# Autodesk Inventor assembly: am14u3LongWithCubeAndWinch
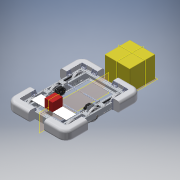
[picture p0: Inventor's stored thumbnail of the model, 180x180]
Saved by Autodesk Inventor 2018.2 (Build 222227000, 227)
## iProperties
Created: 2018-01-10
Part Number: am14u3LongWithCubeAndWinch
Document SubType Name: Assembly
Designer: steele
Author: steele
## Documents named in this file (5)
- D:\snobotics\CAD-Development\robSteele\2018-FRC\am14u3LongWithCubeAndWinch.iam
- D:\snobotics\CAD-Development\robSteele\2018-FRC\AM14U3 Long with Bumper\DB_DriveBaseLong_AM14U3_Bumpers and Battery Tray.iam
- D:\snobotics\CAD-Development\robSteele\2018-FRC\Field Elements\Cube-GE-18124.ipt
- D:\snobotics\CAD-Development\robSteele\2018-FRC\AluminumPlateForWinch.ipt
- D:\snobotics\CAD-Development\robSteele\2018-FRC\WinchVolume.ipt
## Components (4 placed, 4 different names)
1. DB_DriveBaseLong_AM14U3_Bumpers and Battery Tray:1 [sub-assembly] — Mate:1, Mate:2, Mate:3, Mate:4, Flush:2, Mate:5
2. Cube-GE-18124:1 — Mate:1, Flush:1, Mate:2
3. AluminumPlateForWinch:1 — Mate:3, Mate:4, Flush:2, Mate:6, Flush:3
4. WinchVolume:1 — Mate:5, Mate:6, Flush:3
## Relationships (9: Mate 6, Flush 3)
- Mate:1: DB_DriveBaseLong_AM14U3_Bumpers and Battery Tray:1 ↔ Cube-GE-18124:1
- Flush:1: Cube-GE-18124:1
- Mate:2 (152.4 mm): DB_DriveBaseLong_AM14U3_Bumpers and Battery Tray:1 ↔ Cube-GE-18124:1
- Mate:3 (25.4 mm): DB_DriveBaseLong_AM14U3_Bumpers and Battery Tray:1 ↔ AluminumPlateForWinch:1
- Mate:4 (25.4 mm): DB_DriveBaseLong_AM14U3_Bumpers and Battery Tray:1 ↔ AluminumPlateForWinch:1
- Flush:2: DB_DriveBaseLong_AM14U3_Bumpers and Battery Tray:1 ↔ AluminumPlateForWinch:1
- Mate:5: DB_DriveBaseLong_AM14U3_Bumpers and Battery Tray:1 ↔ WinchVolume:1
- Mate:6: AluminumPlateForWinch:1 ↔ WinchVolume:1
- Flush:3: AluminumPlateForWinch:1 ↔ WinchVolume:1
